# Autodesk Inventor assembly: ToASI-4
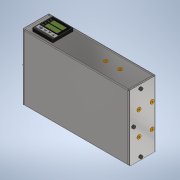
[picture p0: Inventor's stored thumbnail of the model, 180x180]
Saved by Autodesk Inventor 2020.3 (Build 243373000, 373)
## iProperties
Created: 2020-08-01
Part Number: ToASI-4
Document SubType Name: Assembly
Designer: Bruno
Author: Bruno
## Documents named in this file (4)
- C:\Users\Bruno\Desktop\Github\CAD\Inventor\For ASI\ToASI-4.iam
- C:\Users\Bruno\Desktop\Github\CAD\Inventor\For ASI\ToASI-3.iam
- C:\Users\Bruno\Desktop\Github\CAD\Inventor\For ASI\ToASI-2.iam
- C:\Users\Bruno\Desktop\Github\CAD\Inventor\Heater-Box\Box-Disk\DIN912 M4x0.7x10-8.8 socket head screw.ipt
## Components (12 placed, 3 different names)
1. ToASI-3:1 [sub-assembly] — Mate:1, Mate:2, Insert:1
2. ToASI-2:1 [sub-assembly] — Mate:1, Mate:2, Insert:1, Cylindrical:1, Cylindrical:2, Cylindrical:3, Cylindrical:4, Cylindrical:5, Cylindrical:6, Cylindrical:7, Cylindrical:8, Cylindrical:9, Cylindrical:10
3. DIN912 M4x0.7x10-8.8 socket head screw:1 — Cylindrical:10
4. DIN912 M4x0.7x10-8.8 socket head screw:2 — Cylindrical:9
5. DIN912 M4x0.7x10-8.8 socket head screw:3 — Cylindrical:8
6. DIN912 M4x0.7x10-8.8 socket head screw:4 — Cylindrical:3
7. DIN912 M4x0.7x10-8.8 socket head screw:5 — Cylindrical:2
8. DIN912 M4x0.7x10-8.8 socket head screw:6 — Cylindrical:1
9. DIN912 M4x0.7x10-8.8 socket head screw:7 — Cylindrical:4
10. DIN912 M4x0.7x10-8.8 socket head screw:8 — Cylindrical:5
11. DIN912 M4x0.7x10-8.8 socket head screw:9 — Cylindrical:7
12. DIN912 M4x0.7x10-8.8 socket head screw:10 — Cylindrical:6
## Relationships (13: CylindricalJoint 10, Mate 2, Insert 1)
- Mate:1: ToASI-3:1 ↔ ToASI-2:1
- Mate:2: ToASI-3:1 ↔ ToASI-2:1
- Insert:1: ToASI-3:1 ↔ ToASI-2:1
- Cylindrical:1: ToASI-2:1 ↔ DIN912 M4x0.7x10-8.8 socket head screw:6
- Cylindrical:2: ToASI-2:1 ↔ DIN912 M4x0.7x10-8.8 socket head screw:5
- Cylindrical:3: ToASI-2:1 ↔ DIN912 M4x0.7x10-8.8 socket head screw:4
- Cylindrical:4: ToASI-2:1 ↔ DIN912 M4x0.7x10-8.8 socket head screw:7
- Cylindrical:5: ToASI-2:1 ↔ DIN912 M4x0.7x10-8.8 socket head screw:8
- Cylindrical:6: ToASI-2:1 ↔ DIN912 M4x0.7x10-8.8 socket head screw:10
- Cylindrical:7: ToASI-2:1 ↔ DIN912 M4x0.7x10-8.8 socket head screw:9
- Cylindrical:8: ToASI-2:1 ↔ DIN912 M4x0.7x10-8.8 socket head screw:3
- Cylindrical:9: ToASI-2:1 ↔ DIN912 M4x0.7x10-8.8 socket head screw:2
- Cylindrical:10: ToASI-2:1 ↔ DIN912 M4x0.7x10-8.8 socket head screw:1
